# Autodesk Inventor assembly: frame
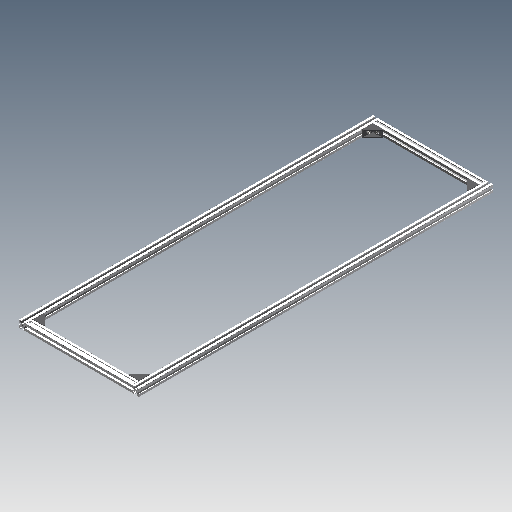
[picture p0: Inventor's stored thumbnail of the model, 512x512]
Saved by Autodesk Inventor 2018 (Build 220112000, 112)
## iProperties
Created: 2017-03-01
Part Number: frame
Document SubType Name: Assembly
Designer: sawaiz
Author: sawaiz
## Documents named in this file (5)
- C:\Users\sawaiz\OneDrive\projects\sPhenixTileTestStand\frame\base.iam
- C:\Users\sawaiz\OneDrive\projects\sPhenixTileTestStand\frame\hfs5-2020Width.ipt
- C:\Users\sawaiz\OneDrive\projects\sPhenixTileTestStand\hardware\angleBracket.iam
- C:\Users\sawaiz\OneDrive\projects\sPhenixTileTestStand\frame\hfs5-2020Depth.ipt
- C:\Users\sawaiz\OneDrive\projects\sPhenixTileTestStand\sPhenixTileTestStand.xlsx
## Components (8 placed, 3 different names)
1. hfs5-2020Width:1 — Mate:8, Mate:9, Flush:14, Flush:15, Flush:16, Symmetry:2, Flush:21, Flush:22, Flush:24
2. angleBracket:1 [sub-assembly] — Angle:7, Flush:9, Flush:10, Mate:8, Flush:11, Flush:12, Flush:16, Symmetry:3, Flush:23, Mate:12
3. angleBracket:2 [sub-assembly] — Flush:10, Flush:12, Flush:13, Flush:17, Mate:10, Flush:18
4. angleBracket:3 [sub-assembly] — Flush:13, Mate:11, Flush:19, Symmetry:1, Symmetry:3, Flush:20
5. angleBracket:4 [sub-assembly] — Angle:7, Flush:9, Mate:9, Flush:11, Flush:14, Flush:15, Symmetry:1, Flush:20, Mate:13
6. hfs5-2020Width:2 — Flush:17, Mate:10, Flush:18, Mate:11, Flush:19, Symmetry:2, Flush:25
7. hfs5-2020Depth:1 — Flush:21, Flush:24, Mate:13, Flush:25
8. hfs5-2020Depth:2 — Flush:22, Flush:23, Mate:12
## Relationships (27: Flush 17, Mate 6, Symmetry 3, Angle 1)
- Angle:7 (0 deg): angleBracket:1 ↔ angleBracket:4
- Flush:9: angleBracket:1 ↔ angleBracket:4
- Flush:10: angleBracket:1 ↔ angleBracket:2
- Mate:8: hfs5-2020Width:1 ↔ angleBracket:1
- Mate:9: hfs5-2020Width:1 ↔ angleBracket:4
- Flush:11: angleBracket:1 ↔ angleBracket:4
- Flush:12: angleBracket:1 ↔ angleBracket:2
- Flush:13: angleBracket:2 ↔ angleBracket:3
- Flush:14: hfs5-2020Width:1 ↔ angleBracket:4
- Flush:15: hfs5-2020Width:1 ↔ angleBracket:4
- Flush:16: hfs5-2020Width:1 ↔ angleBracket:1
- Flush:17: angleBracket:2 ↔ hfs5-2020Width:2
- Mate:10: angleBracket:2 ↔ hfs5-2020Width:2
- Flush:18: angleBracket:2 ↔ hfs5-2020Width:2
- Mate:11: angleBracket:3 ↔ hfs5-2020Width:2
- Flush:19: angleBracket:3 ↔ hfs5-2020Width:2
- Symmetry:1: angleBracket:3 ↔ angleBracket:4
- Symmetry:2: hfs5-2020Width:1 ↔ hfs5-2020Width:2
- Symmetry:3: angleBracket:1 ↔ angleBracket:3
- Flush:20: angleBracket:3 ↔ angleBracket:4
- Flush:21: hfs5-2020Width:1 ↔ hfs5-2020Depth:1
- Flush:22: hfs5-2020Width:1 ↔ hfs5-2020Depth:2
- Flush:23: angleBracket:1 ↔ hfs5-2020Depth:2
- Flush:24: hfs5-2020Width:1 ↔ hfs5-2020Depth:1
- Mate:12: angleBracket:1 ↔ hfs5-2020Depth:2
- Mate:13: angleBracket:4 ↔ hfs5-2020Depth:1
- Flush:25: hfs5-2020Width:2 ↔ hfs5-2020Depth:1
## Named parameters: plateWidth = 300 mm, plateDepth = 1000 mm, supportPlateThickness = 6.35 mm, supportPlateWidth = 50 mm, supportPlateFillet = 10 mm, separation = 35 mm, numPanels = 5, centerVerticalRatio = 0.3, height = 150 mm, depth = 1000 mm, width = 300 mm, suppourtPlateLength = 100 mm, acrylicThickness = 3.125 mm
